# Autodesk Inventor assembly: Montagem da Cabeça do CIlindro
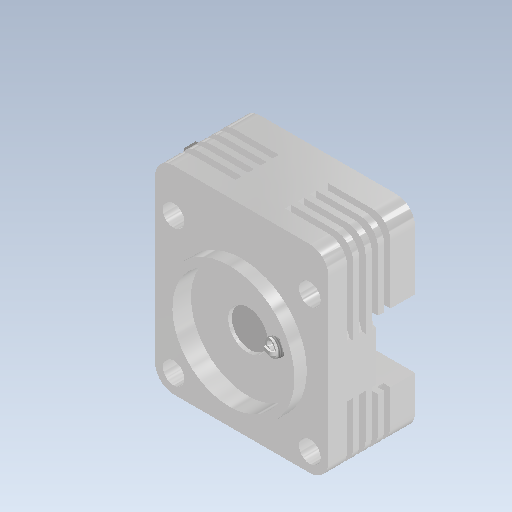
[picture p0: Inventor's stored thumbnail of the model, 512x512]
Saved by Autodesk Inventor 2021 (Build 250183000, 183)
## iProperties
Category: 10
Company: UFABC
Created: 2021-07-26
Document SubType Name: Assembly
Designer: Giovanni
Checked By: Prof. Luis
User Status: 1:5
Author: Giovanni Rodrigues Dias
Title: Montagem da Cabeça do CIlindro
Keywords: 5
Revision Number: 01
## Documents named in this file (12)
- C:\Users\irineu\Documents\Inventor\MotorRadial7\Superior do cilindro 2.iam
- C:\Users\irineu\Documents\Inventor\MotorRadial7\Peça5.2.ipt
- C:\Users\irineu\Documents\Inventor\MotorRadial7\Peça7.ipt
- C:\Users\irineu\Documents\Inventor\MotorRadial7\Peça24.ipt
- C:\Users\irineu\Documents\Inventor\MotorRadial7\Peça17.ipt
- C:\Users\irineu\Documents\Inventor\MotorRadial7\Peça16.ipt
- C:\Users\irineu\Documents\Inventor\MotorRadial7\Peça19 - Copia.ipt
- C:\Users\irineu\Documents\Inventor\MotorRadial7\Peça8.ipt
- C:\Users\irineu\Documents\Inventor\Content Center Files\R2021\pt-BR\DIN 912\DIN 912 - M4 x 0,7 x 20 x 18,25.ipt
- C:\Users\irineu\Documents\Inventor\MotorRadial7\Peça18.ipt
- C:\Users\irineu\Documents\Inventor\Content Center Files\R2021\pt-BR\DIN 6799\DIN 6799 - 8 12.ipt
- C:\Users\irineu\Documents\Inventor\MotorRadial7\Peça45.ipt
## Components (14 placed, 11 different names)
1. Peça5.2:1 — Alinhado:1, Alinhado:2, Coincidente:1, Inserir:1, Coincidente:2, Coincidente:3, Coincidente:6, Coincidente:8, Ângulo:2, Inserir:9
2. Peça7:1 — Inserir:1, Coincidente:5, Inserir:8
3. Peça17:1 — Coincidente:2, Coincidente:3, Coincidente:4
4. Peça45:1 — Inserir:9, Inserir:10
5. Peça24:1 — Inserir:10
6. Peça16:1 — Coincidente:4, Coincidente:5
7. Peça19 - Copia:1 — Coincidente:6, Coincidente:7, Coincidente:8, Coincidente:9, Coincidente:10, Inserir:4, Inserir:5, Coincidente:11
8. Peça8:1 — Coincidente:9, Coincidente:10, Ângulo:2
9. DIN 912 - substituído por DIN EN ISO 4762 M4 x 20:1 — Inserir:4
10. DIN 912 - substituído por DIN EN ISO 4762 M4 x 20:2 — Inserir:5
11. Peça18:1 — Coincidente:11, Coincidente:12, Inserir:6, Inserir:7
12. DIN 6799 8:1 — Inserir:7
13. DIN 6799 8:2 — Inserir:6
14. DIN 6799 8:3 — Inserir:8
## Relationships (23: Mate 12, Insert 8, Flush 2, Angle 1)
- Alinhado:1 [Flush]: Peça5.2:1
- Alinhado:2 [Flush]: Peça5.2:1
- Coincidente:1 [Mate]: Peça5.2:1
- Inserir:1: Peça5.2:1 ↔ Peça7:1
- Coincidente:2 [Mate]: Peça5.2:1 ↔ Peça17:1
- Coincidente:3 [Mate]: Peça5.2:1 ↔ Peça17:1
- Coincidente:4 [Mate]: Peça17:1 ↔ Peça16:1
- Coincidente:5 [Mate]: Peça7:1 ↔ Peça16:1
- Coincidente:6 [Mate]: Peça5.2:1 ↔ Peça19 - Copia:1
- Coincidente:7 [Mate]: Peça19 - Copia:1
- Coincidente:8 [Mate]: Peça5.2:1 ↔ Peça19 - Copia:1
- Coincidente:9 [Mate]: Peça19 - Copia:1 ↔ Peça8:1
- Coincidente:10 [Mate]: Peça19 - Copia:1 ↔ Peça8:1
- Ângulo:2 [Angle] (0 deg): Peça5.2:1 ↔ Peça8:1
- Inserir:4: Peça19 - Copia:1 ↔ DIN 912 - substituído por DIN EN ISO 4762 M4 x 20:1
- Inserir:5: Peça19 - Copia:1 ↔ DIN 912 - substituído por DIN EN ISO 4762 M4 x 20:2
- Coincidente:11 [Mate]: Peça19 - Copia:1 ↔ Peça18:1
- Coincidente:12 [Mate]: Peça18:1
- Inserir:6: Peça18:1 ↔ DIN 6799 8:2
- Inserir:7: Peça18:1 ↔ DIN 6799 8:1
- Inserir:8: Peça7:1 ↔ DIN 6799 8:3
- Inserir:9: Peça5.2:1 ↔ Peça45:1
- Inserir:10: Peça45:1 ↔ Peça24:1
